# Autodesk Inventor assembly: Module
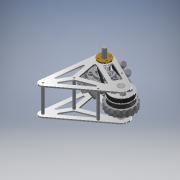
[picture p0: Inventor's stored thumbnail of the model, 180x180]
Saved by Autodesk Inventor 2019.4 (Build 234330000, 330)
## iProperties
Created: 2019-12-31
Part Number: Module
Document SubType Name: Assembly
Designer: Mark
Mass: 2071.33 g
Surface Area: 5536.85 cm^2
Volume: 923.113 cm^3
Density: 2.24385 g/cm^3
Author: Mark
## Documents named in this file (13)
- C:\Users\Mark\Desktop\7738 Helion Engineering\7738-CAD-prep\Butterfly Drive Mk3\Module.iam
- C:\Users\Mark\Desktop\7738 Helion Engineering\7738-CAD-prep\Butterfly Drive Mk3\6_Mecanum_Wheel_Right_217-2586.ipt
- C:\Users\Mark\Desktop\7738 Helion Engineering\7738-CAD-prep\Butterfly Drive Mk3\4_VersaWheel_DT_217-3197.ipt
- C:\Users\Mark\Desktop\7738 Helion Engineering\7738-CAD-prep\Butterfly Drive Mk3\HTD5M 50 Pulley.ipt
- C:\Users\Mark\Desktop\7738 Helion Engineering\7738-CAD-prep\Butterfly Drive Mk3\HTD5M 25 Pulley.ipt
- C:\Users\Mark\Desktop\7738 Helion Engineering\7738-CAD-prep\Butterfly Drive Mk3\HTD5M 93 Belt.ipt
- C:\Users\Mark\Desktop\7738 Helion Engineering\7738-CAD-prep\Butterfly Drive Mk3\Module Plate.ipt
- C:\Users\Mark\Desktop\7738 Helion Engineering\7738-CAD-prep\Butterfly Drive Mk3\F6802.ipt
- C:\Users\Mark\Desktop\7738 Helion Engineering\7738-CAD-prep\Butterfly Drive Mk3\JTW20.ipt
- C:\Users\Mark\Desktop\7738 Helion Engineering\7738-CAD-prep\Butterfly Drive Mk3\16mm ID 4 mm Key Edit1_4_ID_Aluminum_VersaHub_217-3237.ipt
- C:\Users\Mark\Desktop\7738 Helion Engineering\7738-CAD-prep\Butterfly Drive Mk3\Module\Design Accelerator\Shaft1.iam
- C:\Users\Mark\Desktop\7738 Helion Engineering\7738-CAD-prep\Butterfly Drive Mk3\Module\Design Accelerator\Shaft2.iam
- C:\Users\Mark\Desktop\7738 Helion Engineering\7738-CAD-prep\Butterfly Drive Mk3\Module\Design Accelerator\Shaft4.iam
## Components (21 placed, 11 different names)
1. 6_Mecanum_Wheel_Right_217-2586:1 — Mate:1, Flush:1, Mate:4, Mate:5, Mate:30, Mate:31
2. 4_VersaWheel_DT_217-3197:1 — Mate:1, Flush:1, Mate:2, Mate:3, Mate:28, Mate:29
3. HTD5M 50 Pulley:1 — Mate:2, Mate:3, Mate:6, Mate:9
4. HTD5M 25 Pulley:1 — Mate:4, Mate:5, Mate:7, Mate:8, Mate:10, Mate:15
5. HTD5M 93 Belt:1 — Mate:6, Mate:7, Mate:8
6. Module Plate:1 — Mate:9, Mate:10, Mate:11, Mate:12, Mate:13, Mate:14, Mate:15, Mate:16, Mate:23, Mate:27, Mate:33, Flush:4, Mate:38, Mate:40
7. F6802:1 — Mate:11, Mate:12, Mate:17, Mate:22
8. F6802:2 — Mate:13, Mate:14
9. Module Plate:2 — Mate:16, Mate:17, Mate:18, Mate:19, Mate:20, Mate:21, Mate:24, Flush:3, Mate:34, Flush:4, Mate:35, Mate:36, Mate:37, Mate:39
10. F6802:3 — Mate:18, Mate:19, Mate:25, Mate:41
11. F6802:4 — Mate:20, Mate:21, Mate:32
12. JTW20:1 — Mate:22, Mate:23, Mate:27
13. JTW20:2 — Mate:24, Mate:25, Flush:5
14. 16mm ID 5 mm Key Edit1_4_ID_Aluminum_VersaHub_217-3237:1 — Mate:28, Mate:29
15. 16mm ID 4 mm Key Edit1_4_ID_Aluminum_VersaHub_217-3237:2 — Mate:30, Mate:31
16. Shaft:1 [sub-assembly] — Flush:3, Mate:32
17. Shaft:2 [sub-assembly] — Mate:33, Mate:34
18. Shaft:3 [sub-assembly] — Mate:35, Mate:36
19. Shaft:4 [sub-assembly] — Mate:37, Mate:38
20. Shaft:5 [sub-assembly] — Mate:39, Mate:40
21. Shaft:7 [sub-assembly] — Mate:41, Flush:5
## Relationships (44: Mate 40, Flush 4)
- Mate:1 (137.4 mm): 6_Mecanum_Wheel_Right_217-2586:1 ↔ 4_VersaWheel_DT_217-3197:1
- Flush:1: 6_Mecanum_Wheel_Right_217-2586:1 ↔ 4_VersaWheel_DT_217-3197:1
- Mate:2 (10 mm): 4_VersaWheel_DT_217-3197:1 ↔ HTD5M 50 Pulley:1
- Mate:3: 4_VersaWheel_DT_217-3197:1 ↔ HTD5M 50 Pulley:1
- Mate:4 (10 mm): 6_Mecanum_Wheel_Right_217-2586:1 ↔ HTD5M 25 Pulley:1
- Mate:5: 6_Mecanum_Wheel_Right_217-2586:1 ↔ HTD5M 25 Pulley:1
- Mate:6: HTD5M 50 Pulley:1 ↔ HTD5M 93 Belt:1
- Mate:7: HTD5M 25 Pulley:1 ↔ HTD5M 93 Belt:1
- Mate:8 (0.5 mm): HTD5M 25 Pulley:1 ↔ HTD5M 93 Belt:1
- Mate:9: HTD5M 50 Pulley:1 ↔ Module Plate:1
- Mate:10: HTD5M 25 Pulley:1 ↔ Module Plate:1
- Mate:11: Module Plate:1 ↔ F6802:1
- Mate:12: Module Plate:1 ↔ F6802:1
- Mate:13: Module Plate:1 ↔ F6802:2
- Mate:14: Module Plate:1 ↔ F6802:2
- Mate:15 (8 mm): HTD5M 25 Pulley:1 ↔ Module Plate:1
- Mate:16 (100 mm): Module Plate:1 ↔ Module Plate:2
- Mate:17: F6802:1 ↔ Module Plate:2
- Mate:18: Module Plate:2 ↔ F6802:3
- Mate:19: Module Plate:2 ↔ F6802:3
- Mate:20: Module Plate:2 ↔ F6802:4
- Mate:21: Module Plate:2 ↔ F6802:4
- Mate:22: F6802:1 ↔ JTW20:1
- Mate:23: Module Plate:1 ↔ JTW20:1
- Mate:24: Module Plate:2 ↔ JTW20:2
- Mate:25: F6802:3 ↔ JTW20:2
- Mate:27: Module Plate:1 ↔ JTW20:1
- Mate:28: 4_VersaWheel_DT_217-3197:1 ↔ 16mm ID 5 mm Key Edit1_4_ID_Aluminum_VersaHub_217-3237:1
- Mate:29: 4_VersaWheel_DT_217-3197:1 ↔ 16mm ID 5 mm Key Edit1_4_ID_Aluminum_VersaHub_217-3237:1
- Mate:30: 6_Mecanum_Wheel_Right_217-2586:1 ↔ 16mm ID 4 mm Key Edit1_4_ID_Aluminum_VersaHub_217-3237:2
- Mate:31: 6_Mecanum_Wheel_Right_217-2586:1 ↔ 16mm ID 4 mm Key Edit1_4_ID_Aluminum_VersaHub_217-3237:2
- Flush:3: Module Plate:2 ↔ Shaft:1
- Mate:32: F6802:4 ↔ Shaft:1
- Mate:33: Module Plate:1 ↔ Shaft:2
- Mate:34: Module Plate:2 ↔ Shaft:2
- Flush:4: Module Plate:1 ↔ Module Plate:2
- Mate:35: Module Plate:2 ↔ Shaft:3
- Mate:36: Module Plate:2 ↔ Shaft:3
- Mate:37: Module Plate:2 ↔ Shaft:4
- Mate:38: Module Plate:1 ↔ Shaft:4
- Mate:39: Module Plate:2 ↔ Shaft:5
- Mate:40: Module Plate:1 ↔ Shaft:5
- Mate:41: F6802:3 ↔ Shaft:7
- Flush:5: JTW20:2 ↔ Shaft:7
